# Autodesk Inventor assembly: 40mm wheel(with sleeve)
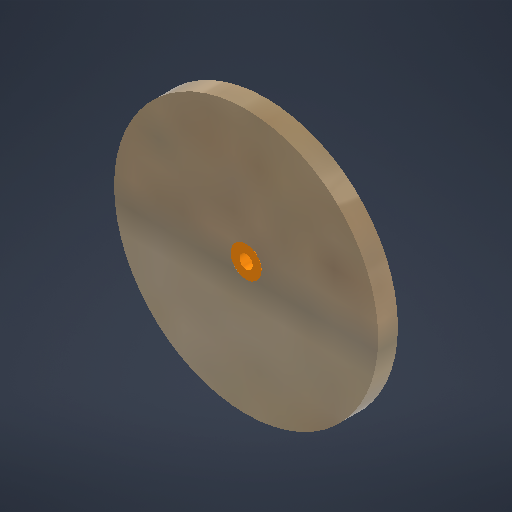
[picture p0: Inventor's stored thumbnail of the model, 512x512]
Saved by Autodesk Inventor 2025.3 (Build 293356030, 356C)
## iProperties
Created: 2025-09-05
Part Number: 40mm wheel(with sleeve)
Document SubType Name: Assembly
Designer: 陳泓任
Author: 陳泓任
## Documents named in this file (3)
- C:\Users\Ou918\機工概論\40mm wheel(with sleeve).iam
- C:\Users\Ou918\機工概論\40mm wheel.ipt
- C:\Users\Ou918\機工概論\sleeve.ipt
## Components (2 placed, 2 different names)
1. 40mm wheel:1 — 插入:1
2. sleeve:1 — 插入:1
## Relationships (1: Insert 1)
- 插入:1 [Insert]: 40mm wheel:1 ↔ sleeve:1
